# Autodesk Inventor assembly: Prototype Assembly
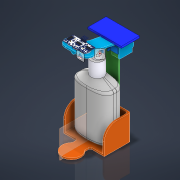
[picture p0: Inventor's stored thumbnail of the model, 180x180]
Saved by Autodesk Inventor 2022 (Build 260153000, 153)
## iProperties
Created: 2021-05-30
Part Number: Prototype Assembly
Document SubType Name: Assembly
Designer: sidsa
Author: sidsa
## Documents named in this file (9)
- D:\My Documents\gIThUB TWS\auto-dispenser\Inventor\Prototype Assembly.iam
- D:\My Documents\gIThUB TWS\auto-dispenser\Inventor\Prototype Base.ipt
- D:\My Documents\gIThUB TWS\auto-dispenser\Inventor\Hand Sanitizer (prototype).ipt
- D:\My Documents\gIThUB TWS\auto-dispenser\Inventor\PreCAD\ServoMotor.ipt
- D:\My Documents\gIThUB TWS\auto-dispenser\Inventor\Vertical Beam Prototype.ipt
- D:\My Documents\gIThUB TWS\auto-dispenser\Inventor\PreCAD\hc-sr04.ipt
- D:\My Documents\gIThUB TWS\auto-dispenser\Inventor\Ultrasonic Gantry.ipt
- D:\My Documents\gIThUB TWS\auto-dispenser\Inventor\PreCAD\Arduino_NANO_CH340.ipt
- D:\My Documents\gIThUB TWS\auto-dispenser\Inventor\PreCAD\solar_panel.ipt
## Components (8 placed, 8 different names)
1. Prototype Base:1 — Mate:1, Mate:3, Flush:1
2. Hand Sanitizer (prototype):1 — Mate:1
3. ServoMotor:1 — Mate:4, Flush:2, Flush:3
4. Vertical Beam Prototype:1 — Mate:3, Flush:1, Mate:4, Flush:2, Flush:3
5. hc-sr04:1 — Mate:7, Angle:1
6. Ultrasonic Gantry:1 — Mate:7, Angle:1, Mate:8
7. Arduino_NANO_CH340:1
8. solar_panel:1 — Mate:8
## Relationships (9: Mate 5, Flush 3, Angle 1)
- Mate:1: Prototype Base:1 ↔ Hand Sanitizer (prototype):1
- Mate:3: Prototype Base:1 ↔ Vertical Beam Prototype:1
- Flush:1: Prototype Base:1 ↔ Vertical Beam Prototype:1
- Mate:4: ServoMotor:1 ↔ Vertical Beam Prototype:1
- Flush:2: ServoMotor:1 ↔ Vertical Beam Prototype:1
- Flush:3: ServoMotor:1 ↔ Vertical Beam Prototype:1
- Mate:7: hc-sr04:1 ↔ Ultrasonic Gantry:1
- Angle:1 (0 deg): hc-sr04:1 ↔ Ultrasonic Gantry:1
- Mate:8: Ultrasonic Gantry:1 ↔ solar_panel:1
